# Autodesk Inventor assembly: SUMA1-20_SUMA1-20_On
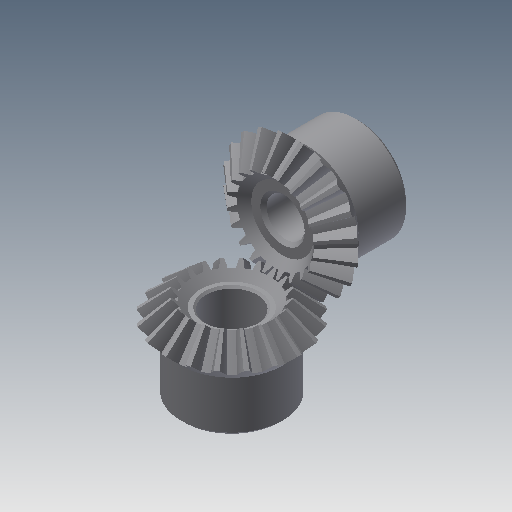
[picture p0: Inventor's stored thumbnail of the model, 512x512]
Saved by Autodesk Inventor 2019.4 (Build 234330000, 330)
## iProperties
Category: PARTsolutions
Company: KHK
Created: 2019-06-11
Part Number: SUMA1-20_SUMA1-20_On
Catalog Web Link: www.cadenas.de
Description: Finished Stainless Steel Miter Gears (SUMA)-
Vendor: KHK
Document SubType Name: Assembly
Designer: psadmin
Manufacturer: KHK
Mass: 4.34126 g
Surface Area: 31.6571 cm^2
Volume: 4.34126 cm^3
Density: 1 g/cm^3
PSOL_IDENT_0: {$CADENAS_DATA\23d-libs\khk\miter_gears\fin_st_steel_miter_gears_suma_asmtab.prj},245 {VTYP=3D},{STY
PSOL_IDENT_1: P=ASSTAB},{NB=SUMA1-20_SUMA1-20_On},{LINA=SUMA1-20_SUMA1-20},{NN=Finished Stainless Steel Miter Gear
PSOL_IDENT_2: s (SUMA)},{DATE=06.06.2019 06:44:34},{GEOMDATE=29.04.2019 10:47:03},{VERSION=},{LINEID=20},{WBVAR=CO
PSOL_IDENT_3: MBINATION,TOOTH},{WBNUMERIC=}  {NB=SUMA1-20_SUMA1-20_On},{LINA=SUMA1-20_SUMA1-20},{KT=DUMMY},{CN=SUM
PSOL_IDENT_4: A1-20},{COMBINATION=2},{M=1.0},{Z=20},{A=6},{B=16},{C=20.0},{D=21.41},{E=20},{F=13.95},{G=10.71},{H=
PSOL_IDENT_5: 8.0},{I=12},{J=5},{K=9.86},{L=49.80},{KYW=0},{KW=0},{KD=0.0},{TDM=4.0},{TS=M4},{S=BT},{PN=SUMA1-20},
PSOL_IDENT_6: {WMF=B3004.WMF},{X=0.5},{Y=0.5},{TSNDM=4},{PPATH=fin_st_steel_miter_gears_suma_asmtpl.prj},{VERS=1},
PSOL_IDENT_7: {CNSORDERNO=SUMA1-20_SUMA1-20},{TOOTH=On}
NN: Finished Stainless Steel Miter Gears (SUMA)
NB: SUMA1-20_SUMA1-20_On
NBSYN: $CNSORDERNO._$TOOTH.
LINA: SUMA1-20_SUMA1-20
CN: SUMA1-20
COMBINATION: Combination
M: 1
Z: 20
A: 6
B: 16
C: 20
D: 21.41
E: 20
F: 13.95
G: 10.71
H: 8
I: 12
J: 5
K: 9.86
L: 49.8
KYW: 0
KW: 0
KD: 0
TDM: 4
TS: M4
S: BT
PN: SUMA1-20
TOOTH: On
SUPPLIER: KHK
ARTICLENO: SUMA1-20_SUMA1-20_On
BOMINFO: SUMA1-20_SUMA1-20
CREATOR: CADENAS GmbH
Title: SUMA1-20_SUMA1-20
Author: Cadenas PARTsolutions
## Documents named in this file (3)
- E:\ロボ研\キャチロボ\キャチロボ2019\アーム2019\KHK_SUMA120SUMA120On\AIS2019\SUMA1-20_SUMA1-20_On.iam
- E:\ロボ研\キャチロボ\キャチロボ2019\アーム2019\KHK_SUMA120SUMA120On\AIS2019\SUMA1-202_On.ipt
- E:\ロボ研\キャチロボ\キャチロボ2019\アーム2019\KHK_SUMA120SUMA120On\AIS2019\SUMA1-201_On.ipt
## Components (2 placed, 2 different names)
1. SUMA1-202_On:1 — メイト:1
2. SUMA1-201_On:1 — メイト:2
## Relationships (2: Mate 2)
- メイト:1 [Mate]: SUMA1-202_On:1
- メイト:2 [Mate]: SUMA1-201_On:1
